# Autodesk Inventor assembly: enclosure_assembly
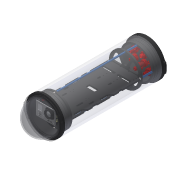
[picture p0: Inventor's stored thumbnail of the model, 180x180]
Saved by Autodesk Inventor 2015 (Build 190159000, 159)
## iProperties
Created: 2016-11-06
Part Number: enclosure_assembly
Document SubType Name: Assembly
Designer: Antonella
Author: Antonella
## Documents named in this file (14)
- C:\Users\Antonella\Documents\Inventor\MicroAUV\Main Enclosure\enclosure_assembly.iam
- C:\Users\Antonella\Documents\Inventor\MicroAUV\Main Enclosure\WTE4-P-TUBE-R1.ipt
- C:\Users\Antonella\Documents\Inventor\MicroAUV\Main Enclosure\WTE4-M-FLANGE-SEAL-R2.ipt
- C:\Users\Antonella\Documents\Inventor\MicroAUV\Main Enclosure\WTE4-M-END-CAP-10X10MM-R1.ipt
- C:\Users\Antonella\Documents\Inventor\MicroAUV\Main Enclosure\WTE4-P-DOME-R1.ipt
- C:\Users\Antonella\Documents\Inventor\MicroAUV\Main Enclosure\ASSEM-ETRAY-R1.ipt
- C:\Users\Antonella\Documents\Inventor\MicroAUV\Penetrators\SWITCH-M-BOLT-10-25-A-R1.ipt
- C:\Users\Antonella\Documents\Inventor\MicroAUV\Penetrators\SWITCH-M-DIAL-10-A-R1.ipt
- C:\Users\Antonella\Documents\Inventor\MicroAUV\Penetrators\PENETRATOR-M-NUT-10-A-R2.ipt
- C:\Users\Antonella\Documents\Inventor\MicroAUV\Penetrators\PENETRATOR-M-BOLT-BLANK-10-25-R2.ipt
- C:\Users\Antonella\Documents\Inventor\MicroAUV\Penetrators\PENETRATOR-M-BOLT-10-25-A-R2.ipt
- C:\Users\Antonella\Documents\Inventor\MicroAUV\Penetrators\VENT-M-BOLT-10-25-A-R3.ipt
- C:\Users\Antonella\Documents\Inventor\MicroAUV\Penetrators\VENT-M-PLUG-10-A-R2.ipt
- C:\Users\Antonella\Documents\Inventor\MicroAUV\GoPro Hero 3 HD Camera\GoPro Hero 3 HD Camera.iam
## Components (29 placed, 13 different names)
1. WTE4-P-TUBE-R1:1 — Mate:1, Mate:2, Mate:3, Mate:4, Mate:6, Mate:10, Mate:11, Mate:12, Mate:13, Flush:1
2. WTE4-M-FLANGE-SEAL-R2:1 — Mate:1, Mate:2, Mate:7, Mate:8, Mate:10
3. WTE4-M-FLANGE-SEAL-R2:2 — Mate:3, Mate:4, Mate:5, Mate:11, Mate:14, Mate:15, Mate:16
4. WTE4-M-END-CAP-10X10MM-R1:1 — Mate:5, Mate:6, Mate:12, Mate:17, Mate:18, Mate:22, Mate:23, Mate:24, Mate:25, Mate:26, Mate:27, Mate:28, Mate:29, Mate:30, Mate:31, Mate:32, Mate:33, Mate:34, Mate:35, Mate:36, Mate:37, Mate:38, Mate:39, Mate:40, Mate:44, Mate:46, Mate:48, Mate:50, Mate:52, Mate:55, Mate:57, Mate:59, Mate:61
5. WTE4-P-DOME-R1:1 — Mate:7, Mate:8, Mate:13
6. ASSEM-ETRAY-R1:1 — Mate:14, Mate:15, Mate:16, Mate:62
7. GoPro Hero 3 HD Camera:1 [sub-assembly] — Mate:62, Flush:1
8. SWITCH-M-BOLT-10-25-A-R1:1 — Mate:17, Mate:18, Mate:19, Mate:20, Mate:21
9. SWITCH-M-DIAL-10-A-R1:1 — Mate:19, Mate:20
10. PENETRATOR-M-BOLT-BLANK-10-25-R2:1 — Mate:25, Mate:26, Mate:51
11. PENETRATOR-M-BOLT-BLANK-10-25-R2:2 — Mate:29, Mate:30, Mate:58
12. PENETRATOR-M-BOLT-BLANK-10-25-R2:3 — Mate:23, Mate:24, Mate:56
13. PENETRATOR-M-BOLT-BLANK-10-25-R2:4 — Mate:27, Mate:28, Mate:60
14. PENETRATOR-M-BOLT-10-25-A-R2:1 — Mate:37, Mate:38, Mate:49
15. PENETRATOR-M-BOLT-10-25-A-R2:2 — Mate:35, Mate:36, Mate:43
16. PENETRATOR-M-BOLT-10-25-A-R2:3 — Mate:33, Mate:34, Mate:45
17. PENETRATOR-M-BOLT-10-25-A-R2:4 — Mate:31, Mate:32, Mate:47
18. VENT-M-BOLT-10-25-A-R3:1 — Mate:39, Mate:40, Mate:41, Mate:42, Mate:54
19. VENT-M-PLUG-10-A-R2:1 — Mate:41, Mate:42
20. PENETRATOR-M-NUT-10-A-R2:1 — Mate:21, Mate:22
21. PENETRATOR-M-NUT-10-A-R2:2 — Mate:45, Mate:46
22. PENETRATOR-M-NUT-10-A-R2:3 — Mate:47, Mate:48
23. PENETRATOR-M-NUT-10-A-R2:4 — Mate:43, Mate:44
24. PENETRATOR-M-NUT-10-A-R2:5 — Mate:54, Mate:55
25. PENETRATOR-M-NUT-10-A-R2:7 — Mate:49, Mate:50
26. PENETRATOR-M-NUT-10-A-R2:8 — Mate:51, Mate:52
27. PENETRATOR-M-NUT-10-A-R2:9 — Mate:56, Mate:57
28. PENETRATOR-M-NUT-10-A-R2:10 — Mate:58, Mate:59
29. PENETRATOR-M-NUT-10-A-R2:11 — Mate:60, Mate:61
## Relationships (61: Mate 60, Flush 1)
- Mate:1: WTE4-P-TUBE-R1:1 ↔ WTE4-M-FLANGE-SEAL-R2:1
- Mate:2: WTE4-P-TUBE-R1:1 ↔ WTE4-M-FLANGE-SEAL-R2:1
- Mate:3: WTE4-P-TUBE-R1:1 ↔ WTE4-M-FLANGE-SEAL-R2:2
- Mate:4: WTE4-P-TUBE-R1:1 ↔ WTE4-M-FLANGE-SEAL-R2:2
- Mate:5: WTE4-M-FLANGE-SEAL-R2:2 ↔ WTE4-M-END-CAP-10X10MM-R1:1
- Mate:6: WTE4-P-TUBE-R1:1 ↔ WTE4-M-END-CAP-10X10MM-R1:1
- Mate:7: WTE4-M-FLANGE-SEAL-R2:1 ↔ WTE4-P-DOME-R1:1
- Mate:8: WTE4-M-FLANGE-SEAL-R2:1 ↔ WTE4-P-DOME-R1:1
- Mate:10: WTE4-P-TUBE-R1:1 ↔ WTE4-M-FLANGE-SEAL-R2:1
- Mate:11: WTE4-P-TUBE-R1:1 ↔ WTE4-M-FLANGE-SEAL-R2:2
- Mate:12: WTE4-P-TUBE-R1:1 ↔ WTE4-M-END-CAP-10X10MM-R1:1
- Mate:13: WTE4-P-TUBE-R1:1 ↔ WTE4-P-DOME-R1:1
- Mate:14: WTE4-M-FLANGE-SEAL-R2:2 ↔ ASSEM-ETRAY-R1:1
- Mate:15: WTE4-M-FLANGE-SEAL-R2:2 ↔ ASSEM-ETRAY-R1:1
- Mate:16: WTE4-M-FLANGE-SEAL-R2:2 ↔ ASSEM-ETRAY-R1:1
- Mate:17: WTE4-M-END-CAP-10X10MM-R1:1 ↔ SWITCH-M-BOLT-10-25-A-R1:1
- Mate:18: WTE4-M-END-CAP-10X10MM-R1:1 ↔ SWITCH-M-BOLT-10-25-A-R1:1
- Mate:19: SWITCH-M-BOLT-10-25-A-R1:1 ↔ SWITCH-M-DIAL-10-A-R1:1
- Mate:20: SWITCH-M-BOLT-10-25-A-R1:1 ↔ SWITCH-M-DIAL-10-A-R1:1
- Mate:21: SWITCH-M-BOLT-10-25-A-R1:1 ↔ PENETRATOR-M-NUT-10-A-R2:1
- Mate:22: WTE4-M-END-CAP-10X10MM-R1:1 ↔ PENETRATOR-M-NUT-10-A-R2:1
- Mate:23: WTE4-M-END-CAP-10X10MM-R1:1 ↔ PENETRATOR-M-BOLT-BLANK-10-25-R2:3
- Mate:24: WTE4-M-END-CAP-10X10MM-R1:1 ↔ PENETRATOR-M-BOLT-BLANK-10-25-R2:3
- Mate:25: WTE4-M-END-CAP-10X10MM-R1:1 ↔ PENETRATOR-M-BOLT-BLANK-10-25-R2:1
- Mate:26: WTE4-M-END-CAP-10X10MM-R1:1 ↔ PENETRATOR-M-BOLT-BLANK-10-25-R2:1
- Mate:27: WTE4-M-END-CAP-10X10MM-R1:1 ↔ PENETRATOR-M-BOLT-BLANK-10-25-R2:4
- Mate:28: WTE4-M-END-CAP-10X10MM-R1:1 ↔ PENETRATOR-M-BOLT-BLANK-10-25-R2:4
- Mate:29: WTE4-M-END-CAP-10X10MM-R1:1 ↔ PENETRATOR-M-BOLT-BLANK-10-25-R2:2
- Mate:30: WTE4-M-END-CAP-10X10MM-R1:1 ↔ PENETRATOR-M-BOLT-BLANK-10-25-R2:2
- Mate:31: WTE4-M-END-CAP-10X10MM-R1:1 ↔ PENETRATOR-M-BOLT-10-25-A-R2:4
- Mate:32: WTE4-M-END-CAP-10X10MM-R1:1 ↔ PENETRATOR-M-BOLT-10-25-A-R2:4
- Mate:33: WTE4-M-END-CAP-10X10MM-R1:1 ↔ PENETRATOR-M-BOLT-10-25-A-R2:3
- Mate:34: WTE4-M-END-CAP-10X10MM-R1:1 ↔ PENETRATOR-M-BOLT-10-25-A-R2:3
- Mate:35: WTE4-M-END-CAP-10X10MM-R1:1 ↔ PENETRATOR-M-BOLT-10-25-A-R2:2
- Mate:36: WTE4-M-END-CAP-10X10MM-R1:1 ↔ PENETRATOR-M-BOLT-10-25-A-R2:2
- Mate:37: WTE4-M-END-CAP-10X10MM-R1:1 ↔ PENETRATOR-M-BOLT-10-25-A-R2:1
- Mate:38: WTE4-M-END-CAP-10X10MM-R1:1 ↔ PENETRATOR-M-BOLT-10-25-A-R2:1
- Mate:39: WTE4-M-END-CAP-10X10MM-R1:1 ↔ VENT-M-BOLT-10-25-A-R3:1
- Mate:40: WTE4-M-END-CAP-10X10MM-R1:1 ↔ VENT-M-BOLT-10-25-A-R3:1
- Mate:41: VENT-M-BOLT-10-25-A-R3:1 ↔ VENT-M-PLUG-10-A-R2:1
- Mate:42: VENT-M-BOLT-10-25-A-R3:1 ↔ VENT-M-PLUG-10-A-R2:1
- Mate:43: PENETRATOR-M-BOLT-10-25-A-R2:2 ↔ PENETRATOR-M-NUT-10-A-R2:4
- Mate:44: WTE4-M-END-CAP-10X10MM-R1:1 ↔ PENETRATOR-M-NUT-10-A-R2:4
- Mate:45: PENETRATOR-M-BOLT-10-25-A-R2:3 ↔ PENETRATOR-M-NUT-10-A-R2:2
- Mate:46: WTE4-M-END-CAP-10X10MM-R1:1 ↔ PENETRATOR-M-NUT-10-A-R2:2
- Mate:47: PENETRATOR-M-BOLT-10-25-A-R2:4 ↔ PENETRATOR-M-NUT-10-A-R2:3
- Mate:48: WTE4-M-END-CAP-10X10MM-R1:1 ↔ PENETRATOR-M-NUT-10-A-R2:3
- Mate:49: PENETRATOR-M-BOLT-10-25-A-R2:1 ↔ PENETRATOR-M-NUT-10-A-R2:7
- Mate:50: WTE4-M-END-CAP-10X10MM-R1:1 ↔ PENETRATOR-M-NUT-10-A-R2:7
- Mate:51: PENETRATOR-M-BOLT-BLANK-10-25-R2:1 ↔ PENETRATOR-M-NUT-10-A-R2:8
- Mate:52: WTE4-M-END-CAP-10X10MM-R1:1 ↔ PENETRATOR-M-NUT-10-A-R2:8
- Mate:54: VENT-M-BOLT-10-25-A-R3:1 ↔ PENETRATOR-M-NUT-10-A-R2:5
- Mate:55: WTE4-M-END-CAP-10X10MM-R1:1 ↔ PENETRATOR-M-NUT-10-A-R2:5
- Mate:56: PENETRATOR-M-BOLT-BLANK-10-25-R2:3 ↔ PENETRATOR-M-NUT-10-A-R2:9
- Mate:57: WTE4-M-END-CAP-10X10MM-R1:1 ↔ PENETRATOR-M-NUT-10-A-R2:9
- Mate:58: PENETRATOR-M-BOLT-BLANK-10-25-R2:2 ↔ PENETRATOR-M-NUT-10-A-R2:10
- Mate:59: WTE4-M-END-CAP-10X10MM-R1:1 ↔ PENETRATOR-M-NUT-10-A-R2:10
- Mate:60: PENETRATOR-M-BOLT-BLANK-10-25-R2:4 ↔ PENETRATOR-M-NUT-10-A-R2:11
- Mate:61: WTE4-M-END-CAP-10X10MM-R1:1 ↔ PENETRATOR-M-NUT-10-A-R2:11
- Mate:62: ASSEM-ETRAY-R1:1 ↔ GoPro Hero 3 HD Camera:1
- Flush:1: WTE4-P-TUBE-R1:1 ↔ GoPro Hero 3 HD Camera:1
